# Autodesk Inventor assembly: assembled-antenna
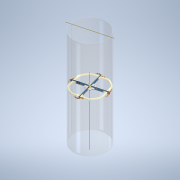
[picture p0: Inventor's stored thumbnail of the model, 180x180]
Saved by Autodesk Inventor 2021 (Build 250183000, 183)
## iProperties
Created: 2020-09-03
Part Number: assembled-antenna
Document SubType Name: Assembly
Designer: dsouthall
Author: dsouthall
## Documents named in this file (7)
- C:\Users\dsouthall\OneDrive - The University of Chicago\Hpol\hpol-prototype\design\Quad-Slot\Model 8 in\assembled-closed-antenna.iam
- C:\Users\dsouthall\OneDrive - The University of Chicago\Hpol\hpol-prototype\design\Quad-Slot\Model 8 in\assembled-feed.iam
- C:\Users\dsouthall\OneDrive - The University of Chicago\Hpol\hpol-prototype\design\Quad-Slot\Model 8 in\source\92141A003_TYPE 18-8 STAINLESS STEEL FLAT WASHER\92141A003_TYPE 18-8 STAINLESS STEEL FLAT WASHER.ipt
- C:\Users\dsouthall\OneDrive - The University of Chicago\Hpol\hpol-prototype\design\Quad-Slot\Model 8 in\source\96877A118_18-8 SS 82 DEG FLAT HEAD PHIL MACHINE SCREW\96877A118_18-8 SS 82 DEG FLAT HEAD PHIL MACHINE SCREW.ipt
- C:\Users\dsouthall\OneDrive - The University of Chicago\Hpol\hpol-prototype\design\Quad-Slot\Model 8 in\source\91841A003_TYPE 18-8 STAINLESS STEEL HEX NUT\91841A003_TYPE 18-8 STAINLESS STEEL HEX NUT.ipt
- C:\Users\dsouthall\OneDrive - The University of Chicago\Hpol\hpol-prototype\design\Quad-Slot\Model 8 in\source\my_faceplate.ipt
- C:\Users\dsouthall\OneDrive - The University of Chicago\Hpol\hpol-prototype\design\Quad-Slot\Model 8 in\source\my can\can_closed.ipt
## Components (28 placed, 6 different names)
1. can_closed:1 — Insert:25, Insert:26, Insert:37, Insert:38, Mate:4, Mate:5, Flush:1, Angle:4, Angle:5
2. my_faceplate:1 — Insert:37, Angle:3
3. my_faceplate:2 — Insert:38, Angle:3
4. assembled-feed:1 [sub-assembly] — Mate:5, Flush:1, Angle:4, Angle:5
5. 92141A003_TYPE 18-8 STAINLESS STEEL FLAT WASHER:12 — Insert:35, Insert:36
6. 91841A003_TYPE 18-8 STAINLESS STEEL HEX NUT:3 — Insert:36
7. 96877A118_18-8 SS 82 DEG FLAT HEAD PHIL MACHINE SCREW:3 — Insert:26, Insert:35
8. 92141A003_TYPE 18-8 STAINLESS STEEL FLAT WASHER:13
9. 91841A003_TYPE 18-8 STAINLESS STEEL HEX NUT:7
10. 96877A118_18-8 SS 82 DEG FLAT HEAD PHIL MACHINE SCREW:7
11. 92141A003_TYPE 18-8 STAINLESS STEEL FLAT WASHER:14
12. 91841A003_TYPE 18-8 STAINLESS STEEL HEX NUT:8
13. 96877A118_18-8 SS 82 DEG FLAT HEAD PHIL MACHINE SCREW:8
14. 92141A003_TYPE 18-8 STAINLESS STEEL FLAT WASHER:15
15. 91841A003_TYPE 18-8 STAINLESS STEEL HEX NUT:9
16. 96877A118_18-8 SS 82 DEG FLAT HEAD PHIL MACHINE SCREW:9
17. 92141A003_TYPE 18-8 STAINLESS STEEL FLAT WASHER:11 — Insert:33, Insert:34
18. 91841A003_TYPE 18-8 STAINLESS STEEL HEX NUT:4 — Insert:34
19. 96877A118_18-8 SS 82 DEG FLAT HEAD PHIL MACHINE SCREW:4 — Insert:25, Insert:33
20. 92141A003_TYPE 18-8 STAINLESS STEEL FLAT WASHER:16
21. 91841A003_TYPE 18-8 STAINLESS STEEL HEX NUT:10
22. 96877A118_18-8 SS 82 DEG FLAT HEAD PHIL MACHINE SCREW:10
23. 92141A003_TYPE 18-8 STAINLESS STEEL FLAT WASHER:17
24. 91841A003_TYPE 18-8 STAINLESS STEEL HEX NUT:11
25. 96877A118_18-8 SS 82 DEG FLAT HEAD PHIL MACHINE SCREW:11
26. 92141A003_TYPE 18-8 STAINLESS STEEL FLAT WASHER:18
27. 91841A003_TYPE 18-8 STAINLESS STEEL HEX NUT:12
28. 96877A118_18-8 SS 82 DEG FLAT HEAD PHIL MACHINE SCREW:12
## Component patterns: (4 elements, first: 92141A003_TYPE 18-8 STAINLESS STEEL FLAT WASHER:12 + 91841A003_TYPE 18-8 STAINLESS STEEL HEX NUT:3 + 96877A118_18-8 SS 82 DEG FLAT HEAD PHIL MACHINE SCREW:3), (4 elements, first: 92141A003_TYPE 18-8 STAINLESS STEEL FLAT WASHER:11 + 91841A003_TYPE 18-8 STAINLESS STEEL HEX NUT:4 + 96877A118_18-8 SS 82 DEG FLAT HEAD PHIL MACHINE SCREW:4)
## Relationships (14: Insert 8, Angle 3, Mate 2, Flush 1)
- Insert:25: can_closed:1 ↔ 96877A118_18-8 SS 82 DEG FLAT HEAD PHIL MACHINE SCREW:4
- Insert:26: can_closed:1 ↔ 96877A118_18-8 SS 82 DEG FLAT HEAD PHIL MACHINE SCREW:3
- Insert:33 (-2.54 mm): 92141A003_TYPE 18-8 STAINLESS STEEL FLAT WASHER:11 ↔ 96877A118_18-8 SS 82 DEG FLAT HEAD PHIL MACHINE SCREW:4
- Insert:34: 92141A003_TYPE 18-8 STAINLESS STEEL FLAT WASHER:11 ↔ 91841A003_TYPE 18-8 STAINLESS STEEL HEX NUT:4
- Insert:35 (-2.54 mm): 92141A003_TYPE 18-8 STAINLESS STEEL FLAT WASHER:12 ↔ 96877A118_18-8 SS 82 DEG FLAT HEAD PHIL MACHINE SCREW:3
- Insert:36: 92141A003_TYPE 18-8 STAINLESS STEEL FLAT WASHER:12 ↔ 91841A003_TYPE 18-8 STAINLESS STEEL HEX NUT:3
- Insert:37: can_closed:1 ↔ my_faceplate:1
- Insert:38 (-9.652 mm): can_closed:1 ↔ my_faceplate:2
- Angle:3 (0 deg): my_faceplate:1 ↔ my_faceplate:2
- Mate:4 (600 mm): can_closed:1
- Mate:5: can_closed:1 ↔ assembled-feed:1
- Flush:1 (-299.2 mm): can_closed:1 ↔ assembled-feed:1
- Angle:4 (0 deg): can_closed:1 ↔ assembled-feed:1
- Angle:5 (0 deg): can_closed:1 ↔ assembled-feed:1
